# Autodesk Inventor assembly: !second_stage
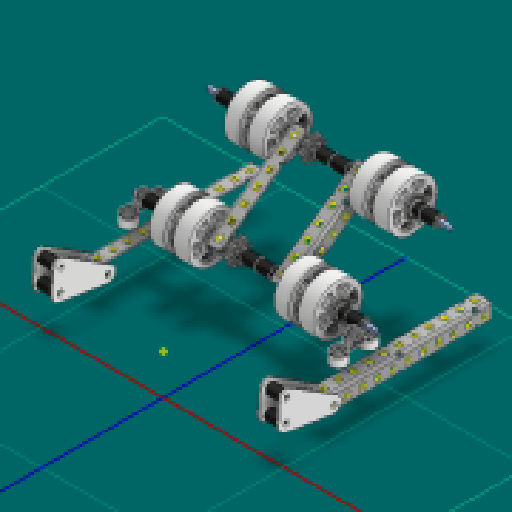
[picture p0: Inventor's stored thumbnail of the model, 512x512]
Saved by Autodesk Inventor 2025 (Build 290162000, 162)
## iProperties
Created: 2024-08-19
Part Number: !second_stage
Document SubType Name: Assembly
Designer: averey
Author: averey
## Documents named in this file (5)
- C:\Users\avere\vex_robotics_high_stakes\hardware\cad\ATLAS\intake\second_stage\!second_stage.iam
- C:\Users\avere\vex_robotics_high_stakes\hardware\cad\ATLAS\intake\second_stage\structure\!structure.iam
- C:\Users\avere\vex_robotics_high_stakes\hardware\cad\ATLAS\intake\second_stage\structure_mirrored\!structure_mirrored.iam
- C:\Users\avere\vex_robotics_high_stakes\hardware\cad\VEX-CAD-Inventor\Structure\Angle\Aluminum 1x1\Alu Angle 1x1x7.ipt
- C:\Users\avere\vex_robotics_high_stakes\hardware\cad\ATLAS\intake\first_stage\top_roller.iam
## Components (6 placed, 4 different names)
1. !structure:1 [sub-assembly] — Insert:1, Mate:1, Mate:2, Mate:3, Insert:2, Angle:1
2. !structure_mirrored:1 [sub-assembly] — Insert:1, Mate:1, Insert:3
3. Alu Angle 1x1x7:1 — Insert:2, Mate:4, Angle:1
4. Alu Angle 1x1x7:2 — Insert:3, Mate:4, Insert:5, Insert:6
5. top_roller:1 [sub-assembly] — Insert:6
6. top_roller:2 [sub-assembly] — Insert:5
## Relationships (10: Insert 5, Mate 4, Angle 1)
- Insert:1 (171.45 mm): !structure:1 ↔ !structure_mirrored:1
- Mate:1: !structure:1 ↔ !structure_mirrored:1
- Mate:2: !structure:1
- Mate:3 (85.725 mm): !structure:1
- Insert:2 (57.15 mm): !structure:1 ↔ Alu Angle 1x1x7:1
- Insert:3 (57.15 mm): !structure_mirrored:1 ↔ Alu Angle 1x1x7:2
- Mate:4: Alu Angle 1x1x7:1 ↔ Alu Angle 1x1x7:2
- Angle:1 (155 deg): !structure:1 ↔ Alu Angle 1x1x7:1
- Insert:5: Alu Angle 1x1x7:2 ↔ top_roller:2
- Insert:6: Alu Angle 1x1x7:2 ↔ top_roller:1
